# Autodesk Inventor assembly: Assembly_v2
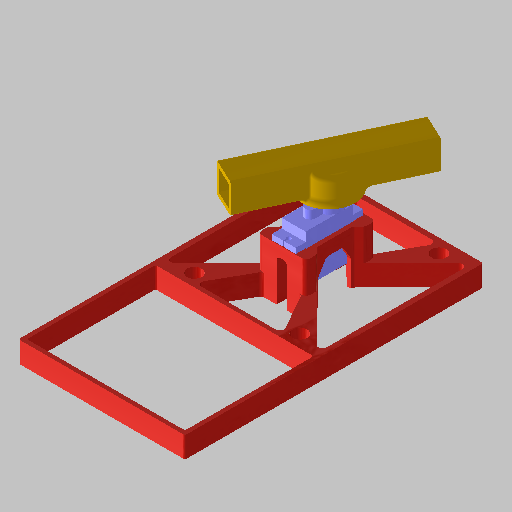
[picture p0: Inventor's stored thumbnail of the model, 512x512]
Saved by Autodesk Inventor 2026.1 (Build 301233020, 233B)
## iProperties
Created: 2025-11-26
Part Number: Assembly_v2
Document SubType Name: Assembly
Designer: samuel
Author: samuel
## Documents named in this file (5)
- E:\Fraunhofer\Design\Assembly_Servo.iam
- E:\Fraunhofer\Design\Servo_holder.ipt
- E:\Fraunhofer\Design\Parts\sg90 micro servo\sg90 micro servo\sg90 micro servo.ipt
- E:\Fraunhofer\Design\Parts\sg90 micro servo\servo_mount_disc.ipt
- E:\Fraunhofer\Design\Servo_magnet.ipt
## Components (4 placed, 4 different names)
1. Servo_holder:1 — Mate:3, Mate:4, Mate:6
2. sg90 micro servo:1 — Mate:3, Mate:4, Mate:6, Mate:7, Mate:8, Mate:12
3. servo_mount_disc:1 — Mate:7, Mate:8, Mate:10, Mate:11
4. Servo_magnet:1 — Mate:10, Mate:11, Mate:12
## Relationships (8: Mate 8)
- Mate:3: Servo_holder:1 ↔ sg90 micro servo:1
- Mate:4: Servo_holder:1 ↔ sg90 micro servo:1
- Mate:6: Servo_holder:1 ↔ sg90 micro servo:1
- Mate:7: sg90 micro servo:1 ↔ servo_mount_disc:1
- Mate:8: sg90 micro servo:1 ↔ servo_mount_disc:1
- Mate:10: servo_mount_disc:1 ↔ Servo_magnet:1
- Mate:11: servo_mount_disc:1 ↔ Servo_magnet:1
- Mate:12: sg90 micro servo:1 ↔ Servo_magnet:1
